# Autodesk Inventor assembly: circuit_battery
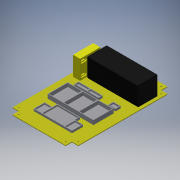
[picture p0: Inventor's stored thumbnail of the model, 180x180]
Saved by Autodesk Inventor 2018.1 (Build 221171000, 171)
## iProperties
Created: 2017-10-03
Part Number: circuit_battery
Material: 一般
Document SubType Name: Assembly
Designer: Kakeru Yamashita
Author: Kakeru Yamashita
## Documents named in this file (8)
- C:\Users\Kakeru Yamashita\Documents\Inventor\Forest_V3\circuit_battery.iam
- C:\Users\Kakeru Yamashita\Documents\Inventor\Forest_V3\arduino.ipt
- C:\Users\Kakeru Yamashita\Documents\Inventor\Forest_V3\motor_driver.ipt
- C:\Users\Kakeru Yamashita\Documents\Inventor\Forest_V3\H8.ipt
- C:\Users\Kakeru Yamashita\Documents\Inventor\Forest_V3\suply_hub.ipt
- C:\Users\Kakeru Yamashita\Documents\Inventor\Forest_V3\dxl_hub.ipt
- C:\Users\Kakeru Yamashita\Documents\Inventor\Forest_remodel\plate_01.ipt
- C:\Users\Kakeru Yamashita\Desktop\terzo tentativo\batterie ecc\Product2.ipt
## Components (11 placed, 7 different names)
1. arduino:1 — メイト:5, フラッシュ:6, メイト:13, メイト:14, フラッシュ:8
2. motor_driver:1 — メイト:1, メイト:10, フラッシュ:1, フラッシュ:5
3. motor_driver:2 — メイト:2, メイト:10, フラッシュ:1, フラッシュ:2, メイト:11
4. motor_driver:3 — メイト:3, フラッシュ:2, メイト:11
5. H8:1 — メイト:4, フラッシュ:4, メイト:13, フラッシュ:8
6. H8:2 — メイト:6, フラッシュ:4, メイト:14
7. suply_hub:1 — メイト:7, メイト:12, フラッシュ:3, フラッシュ:9
8. suply_hub:2 — メイト:8, メイト:12, フラッシュ:3, メイト:17, フラッシュ:10
9. dxl_hub:1 — メイト:9, メイト:17, フラッシュ:10
10. plate_01:1 — メイト:1, メイト:2, メイト:3, メイト:4, メイト:5, メイト:6, メイト:7, メイト:8, メイト:9, フラッシュ:5, フラッシュ:6, フラッシュ:9
11. Product2:1
## Relationships (24: Mate 15, Flush 9)
- メイト:1 [Mate]: motor_driver:1 ↔ plate_01:1
- メイト:2 [Mate]: motor_driver:2 ↔ plate_01:1
- メイト:3 [Mate]: motor_driver:3 ↔ plate_01:1
- メイト:4 [Mate]: H8:1 ↔ plate_01:1
- メイト:5 [Mate]: arduino:1 ↔ plate_01:1
- メイト:6 [Mate]: H8:2 ↔ plate_01:1
- メイト:7 [Mate]: suply_hub:1 ↔ plate_01:1
- メイト:8 [Mate]: suply_hub:2 ↔ plate_01:1
- メイト:9 [Mate]: dxl_hub:1 ↔ plate_01:1
- メイト:10 [Mate]: motor_driver:1 ↔ motor_driver:2
- フラッシュ:1 [Flush]: motor_driver:1 ↔ motor_driver:2
- フラッシュ:2 [Flush]: motor_driver:2 ↔ motor_driver:3
- メイト:11 [Mate]: motor_driver:2 ↔ motor_driver:3
- メイト:12 [Mate]: suply_hub:1 ↔ suply_hub:2
- フラッシュ:3 [Flush]: suply_hub:1 ↔ suply_hub:2
- フラッシュ:4 [Flush]: H8:1 ↔ H8:2
- フラッシュ:5 [Flush] (47 mm): motor_driver:1 ↔ plate_01:1
- フラッシュ:6 [Flush] (101.5 mm): arduino:1 ↔ plate_01:1
- メイト:13 [Mate]: arduino:1 ↔ H8:1
- メイト:14 [Mate]: arduino:1 ↔ H8:2
- フラッシュ:8 [Flush]: arduino:1 ↔ H8:1
- フラッシュ:9 [Flush] (60 mm): suply_hub:1 ↔ plate_01:1
- メイト:17 [Mate] (50 mm): suply_hub:2 ↔ dxl_hub:1
- フラッシュ:10 [Flush]: suply_hub:2 ↔ dxl_hub:1
